# Autodesk Inventor assembly: fork_and_mount
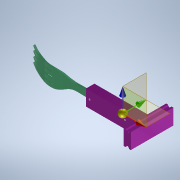
[picture p0: Inventor's stored thumbnail of the model, 180x180]
Saved by Autodesk Inventor 2022 (Build 260153000, 153)
## iProperties
Created: 2022-10-23
Part Number: fork_and_mount
Document SubType Name: Assembly
Designer: Yazawa
Mass: 23.0253 g
Surface Area: 106.018 cm^2
Volume: 13.7015 cm^3
Author: Yazawa
## Documents named in this file (4)
- C:\Users\Yazawa\Documents\GitHub\fork\assembly\fork_and_mount.iam
- C:\Users\Yazawa\Documents\GitHub\fork\parts\fork.ipt
- C:\Users\Yazawa\Documents\GitHub\fork\parts\forkmount.ipt
- C:\Users\Yazawa\Documents\GitHub\fork\parts\BOX-CBF3-8.ipt
## Components (4 placed, 3 different names)
1. fork:1 — メイト:1, メイト:2, メイト:3, メイト:4, メイト:5, メイト:6, メイト:7
2. forkmount:1 — メイト:1, メイト:2, メイト:3
3. BOX-CBF3-8:1 — メイト:4, メイト:7
4. BOX-CBF3-8:2 — メイト:5, メイト:6
## Relationships (7: Mate 7)
- メイト:1 [Mate]: fork:1 ↔ forkmount:1
- メイト:2 [Mate]: fork:1 ↔ forkmount:1
- メイト:3 [Mate]: fork:1 ↔ forkmount:1
- メイト:4 [Mate]: fork:1 ↔ BOX-CBF3-8:1
- メイト:5 [Mate]: fork:1 ↔ BOX-CBF3-8:2
- メイト:6 [Mate]: fork:1 ↔ BOX-CBF3-8:2
- メイト:7 [Mate]: fork:1 ↔ BOX-CBF3-8:1
